# Autodesk Inventor assembly: Assembly
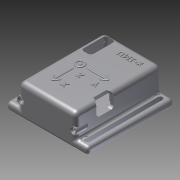
[picture p0: Inventor's stored thumbnail of the model, 180x180]
Saved by Autodesk Inventor 2011 (Build 150239000, 239)
## iProperties
Created: 2011-07-23
Part Number: Assembly
Document SubType Name: Assembly
Designer: Seb Madgwick
Author: Seb Madgwick
## Documents named in this file (3)
- C:\MyFiles\x-io\Products\x-IMU\x-IMU Mechanical\x-IMU v1.3 Housing\x-IMU 1.3 Housing.iam
- C:\MyFiles\x-io\Products\x-IMU\x-IMU Mechanical\x-IMU v1.3 Housing\x-IMU 1.3 Housing - Main.ipt
- C:\MyFiles\x-io\Products\x-IMU\x-IMU Mechanical\x-IMU v1.3 Housing\x-IMU 1.3 Housing - Lid.ipt
## Components (2 placed, 2 different names)
1. x-IMU 1.3 Housing - Main:1 — Insert:1, Insert:2
2. x-IMU 1.3 Housing - Lid:1 — Insert:1, Insert:2
## Relationships (2: Insert 2)
- Insert:1: x-IMU 1.3 Housing - Main:1 ↔ x-IMU 1.3 Housing - Lid:1
- Insert:2: x-IMU 1.3 Housing - Main:1 ↔ x-IMU 1.3 Housing - Lid:1
